# Autodesk Inventor assembly: RS2_Full Assembly
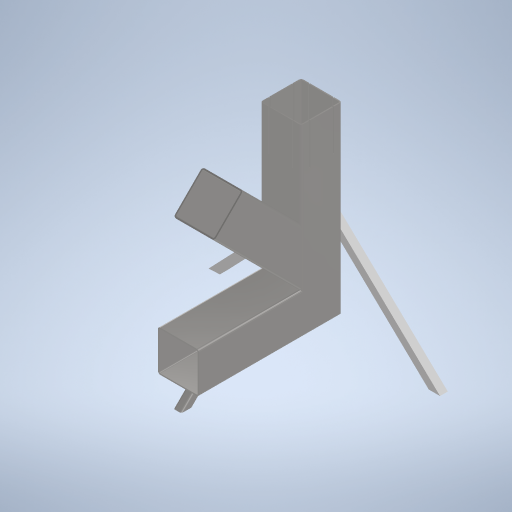
[picture p0: Inventor's stored thumbnail of the model, 512x512]
Saved by Autodesk Inventor 2024.3 (Build 283343000, 343)
## iProperties
Created: 2025-04-13
Part Number: RS2_Full Assembly
Document SubType Name: Assembly
Designer: ajclo
Author: ajclo
## Documents named in this file (4)
- C:\Users\ajclo\OneDrive - Stellenbosch University\Documents\BEng\Year IV\Skripsie\CAD version 2\RS2_Full Assembly.iam
- C:\Users\ajclo\OneDrive - Stellenbosch University\Documents\BEng\Year IV\Skripsie\CAD version 2\RS2_Assembly.iam
- C:\Users\ajclo\OneDrive - Stellenbosch University\Documents\BEng\Year IV\Skripsie\CAD version 2\RS2_TubeFoot.ipt
- C:\Users\ajclo\OneDrive - Stellenbosch University\Documents\BEng\Year IV\Skripsie\CAD version 2\RS2_Tube3rdFoot.iam
## Components (4 placed, 3 different names)
1. RS2_Assembly:1 [sub-assembly] — Mate:3, Mate:4, Flush:2, Mate:5, Mate:6
2. RS2_TubeFoot:1 — Mate:1, Flush:1, Mate:2, Mate:6
3. RS2_TubeFoot:2 — Mate:1, Flush:1, Mate:2, Mate:3, Flush:3
4. RS2_Tube3rdFoot:1 [sub-assembly] — Mate:4, Flush:2, Mate:5, Flush:3
## Relationships (9: Mate 6, Flush 3)
- Mate:1: RS2_TubeFoot:1 ↔ RS2_TubeFoot:2
- Flush:1: RS2_TubeFoot:1 ↔ RS2_TubeFoot:2
- Mate:2: RS2_TubeFoot:1 ↔ RS2_TubeFoot:2
- Mate:3: RS2_Assembly:1 ↔ RS2_TubeFoot:2
- Mate:4: RS2_Assembly:1 ↔ RS2_Tube3rdFoot:1
- Flush:2 (40 mm): RS2_Assembly:1 ↔ RS2_Tube3rdFoot:1
- Mate:5 (-50 mm): RS2_Assembly:1 ↔ RS2_Tube3rdFoot:1
- Flush:3: RS2_TubeFoot:2 ↔ RS2_Tube3rdFoot:1
- Mate:6 (-50 mm): RS2_Assembly:1 ↔ RS2_TubeFoot:1
